# Autodesk Inventor assembly: filament drive
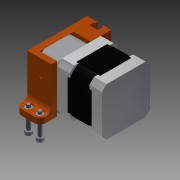
[picture p0: Inventor's stored thumbnail of the model, 180x180]
Saved by Autodesk Inventor 2014 (Build 180170000, 170)
## iProperties
Created: 2013-10-16
Part Number: filament drive
Document SubType Name: Assembly
Designer: employee
Author: employee
## Documents named in this file (8)
- \\GRISTLE\speco\GitHub\ConceptFORGE\Wally\filament drive.iam
- \\GRISTLE\speco\GitHub\ConceptFORGE\Wally\filament drive mount.ipt
- \\GRISTLE\speco\GitHub\ConceptFORGE\Wally\UHMW_block.ipt
- \\GRISTLE\speco\GitHub\ConceptFORGE\Wally\M3x25.ipt
- \\GRISTLE\speco\GitHub\ConceptFORGE\Wally\stepper.ipt
- \\GRISTLE\speco\GitHub\ConceptFORGE\Wally\m3 nut.ipt
- \\GRISTLE\speco\GitHub\ConceptFORGE\Wally\M3x20.ipt
- \\GRISTLE\speco\GitHub\ConceptFORGE\Wally\m4 nut.ipt
## Components (16 placed, 7 different names)
1. filament drive mount:1 — Insert:1, Insert:2, Insert:3, Insert:4, Insert:5, Insert:6, Angle:2, Angle:3, Angle:4, Angle:5, Insert:8, Insert:9, Insert:10, Insert:11, Insert:12, Insert:13, Insert:14, Insert:15, Angle:6, Insert:16
2. UHMW_block:1 — Insert:1, Insert:2, Insert:7, Angle:1
3. M3x25:1 — Insert:4
4. M3x25:2 — Insert:3
5. M3x25:3 — Insert:5
6. M3x25:4 — Insert:6
7. stepper:1 — Insert:7, Angle:1
8. Hex Nut Metric M3 x 0.5:1 — Angle:2, Insert:8
9. Hex Nut Metric M3 x 0.5:2 — Angle:3, Insert:9
10. Hex Nut Metric M3 x 0.5:3 — Angle:4, Insert:10
11. Hex Nut Metric M3 x 0.5:4 — Angle:5, Insert:11
12. Forged Socket Head Cap Screw - Metric M3x0.5 x 20:1 — Insert:12
13. Forged Socket Head Cap Screw - Metric M3x0.5 x 20:2 — Insert:13
14. Forged Socket Head Cap Screw - Metric M3x0.5 x 20:3 — Insert:14
15. Forged Socket Head Cap Screw - Metric M3x0.5 x 20:4 — Insert:15
16. m4 nut:1 — Angle:6, Insert:16
## Relationships (22: Insert 16, Angle 6)
- Insert:1: filament drive mount:1 ↔ UHMW_block:1
- Insert:2: filament drive mount:1 ↔ UHMW_block:1
- Insert:3: filament drive mount:1 ↔ M3x25:2
- Insert:4: filament drive mount:1 ↔ M3x25:1
- Insert:5: filament drive mount:1 ↔ M3x25:3
- Insert:6: filament drive mount:1 ↔ M3x25:4
- Insert:7: UHMW_block:1 ↔ stepper:1
- Angle:1 (0 deg): UHMW_block:1 ↔ stepper:1
- Angle:2 (0 deg): filament drive mount:1 ↔ Hex Nut Metric M3 x 0.5:1
- Angle:3 (0 deg): filament drive mount:1 ↔ Hex Nut Metric M3 x 0.5:2
- Angle:4 (0 deg): filament drive mount:1 ↔ Hex Nut Metric M3 x 0.5:3
- Angle:5 (0 deg): filament drive mount:1 ↔ Hex Nut Metric M3 x 0.5:4
- Insert:8: filament drive mount:1 ↔ Hex Nut Metric M3 x 0.5:1
- Insert:9: filament drive mount:1 ↔ Hex Nut Metric M3 x 0.5:2
- Insert:10: filament drive mount:1 ↔ Hex Nut Metric M3 x 0.5:3
- Insert:11: filament drive mount:1 ↔ Hex Nut Metric M3 x 0.5:4
- Insert:12 (12.5 mm): filament drive mount:1 ↔ Forged Socket Head Cap Screw - Metric M3x0.5 x 20:1
- Insert:13 (12.5 mm): filament drive mount:1 ↔ Forged Socket Head Cap Screw - Metric M3x0.5 x 20:2
- Insert:14 (12.5 mm): filament drive mount:1 ↔ Forged Socket Head Cap Screw - Metric M3x0.5 x 20:3
- Insert:15 (12.5 mm): filament drive mount:1 ↔ Forged Socket Head Cap Screw - Metric M3x0.5 x 20:4
- Angle:6 (0 deg): filament drive mount:1 ↔ m4 nut:1
- Insert:16: filament drive mount:1 ↔ m4 nut:1
